# Autodesk Inventor assembly: a1
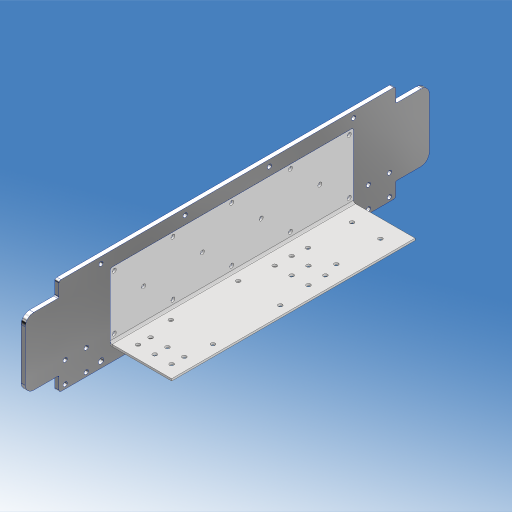
[picture p0: Inventor's stored thumbnail of the model, 512x512]
Saved by Autodesk Inventor 2024 (Build 280153000, 153)
## iProperties
Created: 2024-05-07
Part Number: a1
Document SubType Name: Assembly
Designer: seene
Author: seene
## Documents named in this file (3)
- C:\Users\seene\OneDrive\SBRT\Robocup Rescue\Drive\TestRigs\MainDriveTestrig\a1.iam
- C:\Users\seene\OneDrive\SBRT\Robocup Rescue\Drive\v1\ChassisInterface.ipt
- C:\Users\seene\OneDrive\SBRT\Robocup Rescue\Drive\QuintinCAD\NEMA34_gearbox_sheetMetaMount.ipt
## Components (2 placed, 2 different names)
1. ChassisInterface:1 — Mate:1, Mate:2, Mate:3
2. NEMA34_gearbox_sheetMetaMount:1 — Mate:1, Mate:2, Mate:3
## Relationships (3: Mate 3)
- Mate:1: ChassisInterface:1 ↔ NEMA34_gearbox_sheetMetaMount:1
- Mate:2: ChassisInterface:1 ↔ NEMA34_gearbox_sheetMetaMount:1
- Mate:3: ChassisInterface:1 ↔ NEMA34_gearbox_sheetMetaMount:1
